# Autodesk Inventor assembly: assembly_rotated intake
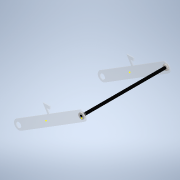
[picture p0: Inventor's stored thumbnail of the model, 180x180]
Saved by Autodesk Inventor 2021.1 (Build 251245000, 245)
## iProperties
Created: 2021-02-27
Part Number: assembly_rotated intake
Document SubType Name: Assembly
Designer: JavDiazV
Author: JavDiazV
## Documents named in this file (4)
- C:\Users\Spade\OneDrive\Documents\t3-cad\CAD\Javier's CAD\assembly_rotated intake.iam
- C:\Users\Spade\OneDrive\Documents\t3-cad\CAD\Javier's CAD\part_0.22 Lexan Intake Arm.ipt
- C:\Users\Spade\OneDrive\Documents\t3-cad\CAD\Javier's CAD\part_18 in. Thundershaft.ipt
- C:\Users\Spade\OneDrive\Documents\t3-cad\CAD\Javier's CAD\part_ Ball Bearing for Thundershaft.ipt
## Components (5 placed, 3 different names)
1. part_0.22 Lexan Intake Arm:1 — Insert:1
2. part_0.22 Lexan Intake Arm:2 — Insert:2
3. part_18 in. Thundershaft:1 — Insert:3, Insert:4
4. part_ Ball Bearing for Thundershaft:1 — Insert:1, Insert:4
5. part_ Ball Bearing for Thundershaft:2 — Insert:2, Insert:3
## Relationships (4: Insert 4)
- Insert:1: part_0.22 Lexan Intake Arm:1 ↔ part_ Ball Bearing for Thundershaft:1
- Insert:2: part_0.22 Lexan Intake Arm:2 ↔ part_ Ball Bearing for Thundershaft:2
- Insert:3: part_18 in. Thundershaft:1 ↔ part_ Ball Bearing for Thundershaft:2
- Insert:4: part_18 in. Thundershaft:1 ↔ part_ Ball Bearing for Thundershaft:1
